# Autodesk Inventor assembly: Durometer_Slide_Fixture
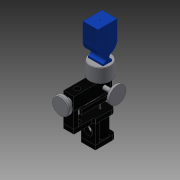
[picture p0: Inventor's stored thumbnail of the model, 180x180]
Saved by Autodesk Inventor 2015 (Build 190159000, 159)
## iProperties
Created: 2014-12-16
Part Number: Durometer_Slide_Fixture
Document SubType Name: Assembly
Designer: amarschn
Author: amarschn
## Documents named in this file (13)
- C:\Users\Drew\Dropbox\Durometer\Durometer_Assembly\Durometer_Slide_Fixture.iam
- C:\Users\Drew\Dropbox\Durometer\Durometer_Assembly\Fixture_Base.ipt
- C:\Users\Drew\Dropbox\Durometer\Durometer_Assembly\Fixture_Base_Support.ipt
- C:\Users\Drew\Dropbox\Durometer\Durometer_Assembly\Fixture_Airpot_Support.ipt
- C:\Users\Drew\Dropbox\Durometer\Durometer_Assembly\Fixture_Airpot_Support_2.ipt
- C:\Users\Drew\Dropbox\Durometer\Durometer_Assembly\Fixture_Airpot_Support_3.ipt
- C:\Users\Drew\Dropbox\Durometer\Durometer_Assembly\Fixture_Airpot.ipt
- C:\Users\Drew\Dropbox\Durometer\Durometer_Assembly\Fixture_Slide_Lock_Plate.ipt
- C:\Users\Drew\Dropbox\Durometer\Durometer_Assembly\Fixture_Weight.ipt
- C:\Users\Drew\Dropbox\Durometer\Durometer_Assembly\Fixture_Knob_1.ipt
- C:\Users\Drew\Dropbox\Durometer\Durometer_Assembly\Fixture_Knob_2.ipt
- C:\Users\Drew\Dropbox\Durometer\Durometer_Assembly\Fixture_Lever.ipt
- C:\Users\Drew\Dropbox\Durometer\Durometer_Assembly\Durometer_Sensor.ipt
## Components (12 placed, 12 different names)
1. Fixture_Base:1 — Mate:1, Flush:1, Flush:2, Mate:2, Mate:8, Mate:9, Angle:1, Mate:11, Mate:12, Mate:13, Mate:14, Mate:15, Mate:16
2. Fixture_Base_Support:1 — Mate:1, Flush:1, Flush:2, Mate:3, Flush:7
3. Fixture_Airpot_Support:1 — Mate:2, Mate:3, Mate:4, Flush:3, Flush:4, Mate:6, Flush:7
4. Fixture_Airpot_Support_2:1 — Mate:5, Flush:5, Flush:6, Mate:7
5. Fixture_Airpot_Support_3:1 — Mate:4, Flush:3, Flush:4, Mate:5, Flush:5, Flush:6
6. Fixture_Airpot:1 — Mate:6, Mate:7
7. Fixture_Slide_Lock_Plate:1 — Mate:10, Angle:1
8. Fixture_Weight:1 — Mate:8, Mate:9, Mate:10, Mate:18, Mate:19
9. Fixture_Knob_1:1 — Mate:13, Mate:14
10. Fixture_Knob_2:1 — Mate:11, Mate:12
11. Fixture_Lever:1 — Mate:15, Mate:16
12. Durometer_Sensor:1 — Mate:18, Mate:19
## Relationships (26: Mate 18, Flush 7, Angle 1)
- Mate:1: Fixture_Base:1 ↔ Fixture_Base_Support:1
- Flush:1: Fixture_Base:1 ↔ Fixture_Base_Support:1
- Flush:2: Fixture_Base:1 ↔ Fixture_Base_Support:1
- Mate:2: Fixture_Base:1 ↔ Fixture_Airpot_Support:1
- Mate:3: Fixture_Base_Support:1 ↔ Fixture_Airpot_Support:1
- Mate:4: Fixture_Airpot_Support:1 ↔ Fixture_Airpot_Support_3:1
- Flush:3: Fixture_Airpot_Support:1 ↔ Fixture_Airpot_Support_3:1
- Flush:4: Fixture_Airpot_Support:1 ↔ Fixture_Airpot_Support_3:1
- Mate:5: Fixture_Airpot_Support_2:1 ↔ Fixture_Airpot_Support_3:1
- Flush:5: Fixture_Airpot_Support_2:1 ↔ Fixture_Airpot_Support_3:1
- Flush:6: Fixture_Airpot_Support_2:1 ↔ Fixture_Airpot_Support_3:1
- Mate:6: Fixture_Airpot_Support:1 ↔ Fixture_Airpot:1
- Mate:7: Fixture_Airpot_Support_2:1 ↔ Fixture_Airpot:1
- Flush:7: Fixture_Base_Support:1 ↔ Fixture_Airpot_Support:1
- Mate:8: Fixture_Base:1 ↔ Fixture_Weight:1
- Mate:9: Fixture_Base:1 ↔ Fixture_Weight:1
- Mate:10: Fixture_Slide_Lock_Plate:1 ↔ Fixture_Weight:1
- Angle:1 (0 deg): Fixture_Base:1 ↔ Fixture_Slide_Lock_Plate:1
- Mate:11: Fixture_Base:1 ↔ Fixture_Knob_2:1
- Mate:12: Fixture_Base:1 ↔ Fixture_Knob_2:1
- Mate:13: Fixture_Base:1 ↔ Fixture_Knob_1:1
- Mate:14: Fixture_Base:1 ↔ Fixture_Knob_1:1
- Mate:15: Fixture_Base:1 ↔ Fixture_Lever:1
- Mate:16: Fixture_Base:1 ↔ Fixture_Lever:1
- Mate:18: Fixture_Weight:1 ↔ Durometer_Sensor:1
- Mate:19: Fixture_Weight:1 ↔ Durometer_Sensor:1
